# Autodesk Inventor assembly: capball lift
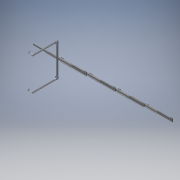
[picture p0: Inventor's stored thumbnail of the model, 180x180]
Saved by Autodesk Inventor 2017 (Build 210142000, 142)
## iProperties
Created: 2016-12-08
Part Number: capball lift
Document SubType Name: Assembly
Designer: Aditya
Author: Aditya
## Documents named in this file (9)
- C:\Users\Aditya\Documents\GitHub\RobotuxCAD\Team Robotux 15-16 Robot Cad Assets\capball lift.iam
- C:\Users\Aditya\Documents\GitHub\RobotuxCAD\Team Robotux 15-16 Robot Cad Assets\Andy Mark Parts\15mm alu ext 14in long.ipt
- C:\Users\Aditya\Documents\GitHub\RobotuxCAD\Team Robotux 15-16 Robot Cad Assets\Andy Mark Parts\15mm alu ext 17in long.ipt
- C:\Users\Aditya\Documents\GitHub\RobotuxCAD\Team Robotux 15-16 Robot Cad Assets\Andy Mark Parts\REV-41-1039.ipt
- C:\Users\Aditya\Documents\GitHub\RobotuxCAD\Team Robotux 15-16 Robot Cad Assets\Andy Mark Parts\REV-41-1038.ipt
- C:\Users\Aditya\Documents\GitHub\RobotuxCAD\Team Robotux 15-16 Robot Cad Assets\Tetrix Parts\tetrix_739103_2012.ipt
- C:\Users\Aditya\Documents\GitHub\RobotuxCAD\Team Robotux 15-16 Robot Cad Assets\Tetrix Parts\tetrix_739387_2013.ipt
- C:\Users\Aditya\Documents\GitHub\RobotuxCAD\Team Robotux 15-16 Robot Cad Assets\Andy Mark Parts\63835A42.iam
- C:\Users\Aditya\Documents\GitHub\RobotuxCAD\Team Robotux 15-16 Robot Cad Assets\Andy Mark Parts\slide plate.ipt
## Components (25 placed, 8 different names)
1. 15mm alu ext 14in long:1 — Mate:1, Flush:1, Flush:2, Mate:3, Flush:5, Flush:12, Mate:10, Mate:16
2. 15mm alu ext 14in long:2 — Mate:2, Flush:3, Flush:4, Flush:7, Mate:5, Flush:9, Mate:7, Flush:13, Mate:15
3. 15mm alu ext 17in long:1 — Mate:1, Flush:1, Flush:2, Mate:2, Flush:3, Flush:4, Flush:6, Mate:4, Flush:8, Flush:10, Mate:6, Flush:11, Mate:8, Mate:9, Flush:14, Mate:28, Flush:27
4. REV-41-1039:1 — Mate:4, Flush:7, Flush:8
5. REV-41-1039:2 — Mate:6, Flush:11, Flush:12
6. REV-41-1039:3 — Mate:5, Flush:9, Flush:10
7. REV-41-1039:4 — Mate:3, Flush:5, Flush:6
8. REV-41-1038:1 — Mate:9, Mate:10, Flush:14
9. REV-41-1038:2 — Mate:7, Mate:8, Flush:13
10. tetrix_739103_2012:1 — Mate:11, Mate:12, Mate:16
11. tetrix_739103_2012:2 — Mate:13, Mate:14, Mate:15
12. tetrix_739387_2013:1 — Mate:13, Mate:14
13. tetrix_739387_2013:2 — Mate:11, Mate:12
14. 63835A42:1 [sub-assembly] — Mate:19, Flush:18, Mate:22, Flush:21, Mate:25, Flush:24
15. 63835A42:2 [sub-assembly] — Mate:20, Flush:19, Mate:21, Flush:20, Mate:28, Flush:27
16. 63835A42:3 [sub-assembly] — Mate:18, Flush:17, Mate:23, Flush:22, Mate:26, Flush:25
17. 63835A42:4 [sub-assembly] — Flush:15, Mate:17, Flush:16, Mate:24, Flush:23, Mate:27, Flush:26
18. slide plate:1 — Flush:15, Mate:17, Flush:16
19. slide plate:2 — Mate:18, Flush:17
20. slide plate:3 — Mate:19, Flush:18
21. slide plate:4 — Mate:20, Flush:19
22. slide plate:5 — Mate:22, Flush:21, Mate:26, Flush:25
23. slide plate:6 — Mate:24, Flush:23
24. slide plate:7 — Mate:23, Flush:22, Mate:27, Flush:26
25. slide plate:8 — Mate:21, Flush:20, Mate:25, Flush:24
## Relationships (55: Mate 28, Flush 27)
- Mate:1: 15mm alu ext 14in long:1 ↔ 15mm alu ext 17in long:1
- Flush:1: 15mm alu ext 14in long:1 ↔ 15mm alu ext 17in long:1
- Flush:2: 15mm alu ext 14in long:1 ↔ 15mm alu ext 17in long:1
- Mate:2: 15mm alu ext 14in long:2 ↔ 15mm alu ext 17in long:1
- Flush:3: 15mm alu ext 14in long:2 ↔ 15mm alu ext 17in long:1
- Flush:4: 15mm alu ext 14in long:2 ↔ 15mm alu ext 17in long:1
- Mate:3: 15mm alu ext 14in long:1 ↔ REV-41-1039:4
- Flush:5: 15mm alu ext 14in long:1 ↔ REV-41-1039:4
- Flush:6: 15mm alu ext 17in long:1 ↔ REV-41-1039:4
- Mate:4: 15mm alu ext 17in long:1 ↔ REV-41-1039:1
- Flush:7: 15mm alu ext 14in long:2 ↔ REV-41-1039:1
- Flush:8: 15mm alu ext 17in long:1 ↔ REV-41-1039:1
- Mate:5: 15mm alu ext 14in long:2 ↔ REV-41-1039:3
- Flush:9: 15mm alu ext 14in long:2 ↔ REV-41-1039:3
- Flush:10: 15mm alu ext 17in long:1 ↔ REV-41-1039:3
- Mate:6: 15mm alu ext 17in long:1 ↔ REV-41-1039:2
- Flush:11: 15mm alu ext 17in long:1 ↔ REV-41-1039:2
- Flush:12: 15mm alu ext 14in long:1 ↔ REV-41-1039:2
- Mate:7: 15mm alu ext 14in long:2 ↔ REV-41-1038:2
- Mate:8: 15mm alu ext 17in long:1 ↔ REV-41-1038:2
- Flush:13: 15mm alu ext 14in long:2 ↔ REV-41-1038:2
- Mate:9: 15mm alu ext 17in long:1 ↔ REV-41-1038:1
- Mate:10: 15mm alu ext 14in long:1 ↔ REV-41-1038:1
- Flush:14: 15mm alu ext 17in long:1 ↔ REV-41-1038:1
- Mate:11: tetrix_739103_2012:1 ↔ tetrix_739387_2013:2
- Mate:12: tetrix_739103_2012:1 ↔ tetrix_739387_2013:2
- Mate:13: tetrix_739103_2012:2 ↔ tetrix_739387_2013:1
- Mate:14: tetrix_739103_2012:2 ↔ tetrix_739387_2013:1
- Mate:15: 15mm alu ext 14in long:2 ↔ tetrix_739103_2012:2
- Mate:16: 15mm alu ext 14in long:1 ↔ tetrix_739103_2012:1
- Flush:15: 63835A42:4 ↔ slide plate:1
- Mate:17: 63835A42:4 ↔ slide plate:1
- Flush:16: 63835A42:4 ↔ slide plate:1
- Mate:18: 63835A42:3 ↔ slide plate:2
- Flush:17: 63835A42:3 ↔ slide plate:2
- Mate:19: 63835A42:1 ↔ slide plate:3
- Flush:18: 63835A42:1 ↔ slide plate:3
- Mate:20: 63835A42:2 ↔ slide plate:4
- Flush:19: 63835A42:2 ↔ slide plate:4
- Mate:21: 63835A42:2 ↔ slide plate:8
- Flush:20: 63835A42:2 ↔ slide plate:8
- Mate:22: 63835A42:1 ↔ slide plate:5
- Flush:21: 63835A42:1 ↔ slide plate:5
- Mate:23: 63835A42:3 ↔ slide plate:7
- Flush:22: 63835A42:3 ↔ slide plate:7
- Mate:24: 63835A42:4 ↔ slide plate:6
- Flush:23: 63835A42:4 ↔ slide plate:6
- Mate:25: 63835A42:1 ↔ slide plate:8
- Flush:24: 63835A42:1 ↔ slide plate:8
- Mate:26: 63835A42:3 ↔ slide plate:5
- Flush:25: 63835A42:3 ↔ slide plate:5
- Mate:27: 63835A42:4 ↔ slide plate:7
- Flush:26: 63835A42:4 ↔ slide plate:7
- Mate:28: 15mm alu ext 17in long:1 ↔ 63835A42:2
- Flush:27: 15mm alu ext 17in long:1 ↔ 63835A42:2
